# Autodesk Inventor assembly: PPUMPASS
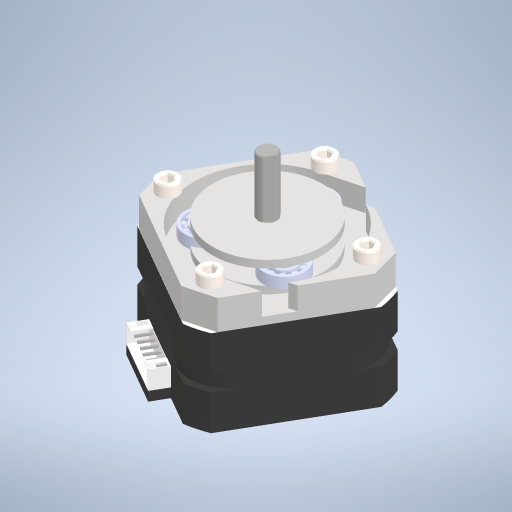
[picture p0: Inventor's stored thumbnail of the model, 512x512]
Saved by Autodesk Inventor 2023 (Build 270158000, 158)
## iProperties
Created: 2022-12-06
Part Number: PPUMPASS
Document SubType Name: Assembly
Designer: Owner
Author: Owner
## Documents named in this file (6)
- C:\Users\Owner\Desktop\ppump\PPUMPASS.iam
- C:\Users\Owner\Documents\Inventor\bearing -5-11-3.ipt
- C:\Users\Owner\Desktop\ppump\insert.ipt
- C:\Users\Owner\Desktop\ppump\Imported Components\Motor a pasos Nema 17 17HS4023\Motor a pasos Nema 17 17HS4023.iam
- C:\Users\Owner\Desktop\ppump\Pumphousing.ipt
- C:\Users\Owner\Desktop\ppump\M3x8.ipt
## Components (11 placed, 5 different names)
1. bearing -5-11-3:1 — Rigid:3
2. insert:1 — Mate:1, Mate:2, Mate:3, Mate:4, Mate:5, Rigid:2, Mate:6
3. Motor a pasos Nema 17 17HS4023:1 [sub-assembly] — Rigid:1, Mate:2, Mate:3, Cylindrical:1
4. Pumphousing:1 — Rigid:1, Mate:1, Rotational:1, Rotational:2, Rotational:3, Rotational:4
5. insert:2 — Cylindrical:1, Mate:4, Mate:5, Rigid:3
6. M3x8:1 — Rotational:1
7. M3x8:2 — Rotational:2
8. M3x8:3 — Rotational:3
9. M3x8:4 — Rotational:4
10. bearing -5-11-3:2 — Rigid:2
11. bearing -5-11-3:3 — Mate:6
## Relationships (14: Mate 6, RevoluteJoint 4, WeldJoint 3, CylindricalJoint 1)
- Rigid:1 [WeldJoint]: Motor a pasos Nema 17 17HS4023:1 ↔ Pumphousing:1
- Mate:1: insert:1 ↔ Pumphousing:1
- Mate:2: insert:1 ↔ Motor a pasos Nema 17 17HS4023:1
- Mate:3: insert:1 ↔ Motor a pasos Nema 17 17HS4023:1
- Cylindrical:1: Motor a pasos Nema 17 17HS4023:1 ↔ insert:2
- Mate:4: insert:1 ↔ insert:2
- Mate:5: insert:1 ↔ insert:2
- Rigid:2 [WeldJoint] (-1 mm): insert:1 ↔ bearing -5-11-3:2
- Mate:6: insert:1 ↔ bearing -5-11-3:3
- Rigid:3 [WeldJoint]: bearing -5-11-3:1 ↔ insert:2
- Rotational:1 [RevoluteJoint]: Pumphousing:1 ↔ M3x8:1
- Rotational:2 [RevoluteJoint]: Pumphousing:1 ↔ M3x8:2
- Rotational:3 [RevoluteJoint]: Pumphousing:1 ↔ M3x8:3
- Rotational:4 [RevoluteJoint]: Pumphousing:1 ↔ M3x8:4
